# Autodesk Inventor assembly: Battery Cage and Spring Plate
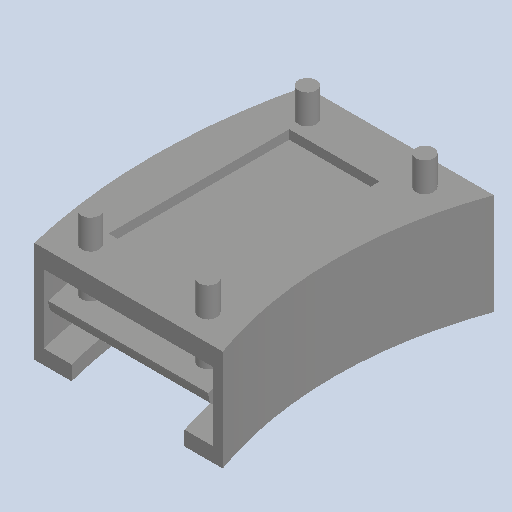
[picture p0: Inventor's stored thumbnail of the model, 512x512]
Saved by Autodesk Inventor 2023 (Build 270158000, 158)
## iProperties
Created: 2023-02-15
Part Number: Battery Cage and Spring Plate
Document SubType Name: Assembly
Designer: mihal
Mass: 157.198 g
Surface Area: 1142.15 cm^2
Volume: 380.163 cm^3
Density: 0.4135 g/cm^3
Author: mihal
## Documents named in this file (3)
- C:\Users\mihal\Desktop\12a th Assembly\Battery Cage and Spring Plate.iam
- C:\Users\mihal\Desktop\12a th Assembly\Battery Cage Second Iteration.ipt
- C:\Users\mihal\Desktop\12a th Assembly\Battery Cage Spring Plate Second Iteration.ipt
## Components (2 placed, 2 different names)
1. Battery Cage Second Iteration:1 — Mate:1, Mate:2
2. Battery Cage Spring Plate Second Iteration:1 — Mate:1, Mate:2
## Relationships (2: Mate 2)
- Mate:1: Battery Cage Second Iteration:1 ↔ Battery Cage Spring Plate Second Iteration:1
- Mate:2: Battery Cage Second Iteration:1 ↔ Battery Cage Spring Plate Second Iteration:1
